# Autodesk Inventor assembly: cable-hanger-hook
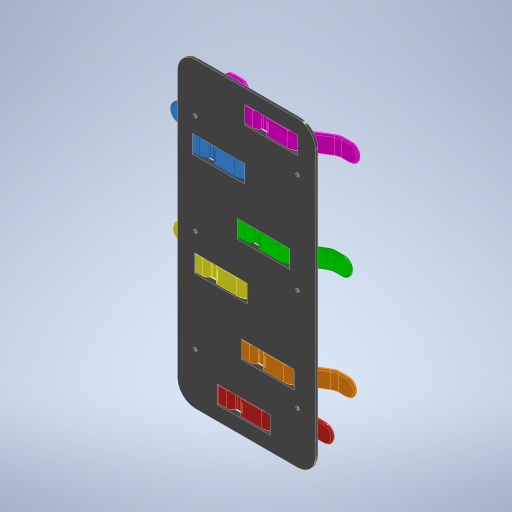
[picture p0: Inventor's stored thumbnail of the model, 512x512]
Saved by Autodesk Inventor 2023 (Build 270158030, 158C)
## iProperties
Created: 2024-09-23
Part Number: cable-hanger-hook
Document SubType Name: Assembly
Designer: Imogen Heard
Author: Imogen Heard
## Documents named in this file (3)
- C:\Users\dheard\Documents\0004-inventor\3D-CAD-main\cable-hanger\cable-hanger-hook.iam
- C:\Users\dheard\Documents\0004-inventor\3D-CAD-main\cable-hanger\cable-hanger.ipt
- C:\Users\dheard\Documents\0004-inventor\3D-CAD-main\cable-hanger\backplate-0.ipt
## Components (7 placed, 2 different names)
1. cable-hanger:1 — Flush:1
2. backplate-0:1 — Flush:1, Mate:1, Mate:2, Mate:3, Mate:4, Mate:5, Mate:6, Mate:7, Mate:8, Mate:9, Mate:10, Mate:11, Mate:12, Mate:13, Mate:14, Mate:15, Mate:16
3. cable-hanger:2 — Mate:1, Mate:13, Mate:14
4. cable-hanger:3 — Mate:2, Mate:12, Mate:15
5. cable-hanger:4 — Mate:3, Mate:11, Mate:16
6. cable-hanger:5 — Mate:4, Mate:7, Mate:9, Mate:10
7. cable-hanger:6 — Mate:5, Mate:6, Mate:8
## Relationships (17: Mate 16, Flush 1)
- Flush:1: cable-hanger:1 ↔ backplate-0:1
- Mate:1: backplate-0:1 ↔ cable-hanger:2
- Mate:2: backplate-0:1 ↔ cable-hanger:3
- Mate:3: backplate-0:1 ↔ cable-hanger:4
- Mate:4: backplate-0:1 ↔ cable-hanger:5
- Mate:5: backplate-0:1 ↔ cable-hanger:6
- Mate:6: backplate-0:1 ↔ cable-hanger:6
- Mate:7: backplate-0:1 ↔ cable-hanger:5
- Mate:8: backplate-0:1 ↔ cable-hanger:6
- Mate:9: backplate-0:1 ↔ cable-hanger:5
- Mate:10: backplate-0:1 ↔ cable-hanger:5
- Mate:11: backplate-0:1 ↔ cable-hanger:4
- Mate:12: backplate-0:1 ↔ cable-hanger:3
- Mate:13: backplate-0:1 ↔ cable-hanger:2
- Mate:14: backplate-0:1 ↔ cable-hanger:2
- Mate:15: backplate-0:1 ↔ cable-hanger:3
- Mate:16: backplate-0:1 ↔ cable-hanger:4
